# Autodesk Inventor assembly: KB33-046-001 - Ходовая часть
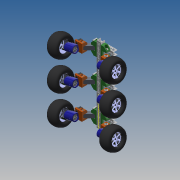
[picture p0: Inventor's stored thumbnail of the model, 180x180]
Saved by Autodesk Inventor 2020 (Build 240168000, 168)
## iProperties
Created: 2021-06-08
Part Number: KB33-046-001 - Ходовая часть
Material: Типовые
Document SubType Name: Assembly
Designer: Петров Иван
Mass: 8557.92 g
Surface Area: 14903.5 cm^2
Volume: 8211.85 cm^3
Density: 1.04214 g/cm^3
Author: Петров Иван
## Documents named in this file (6)
- E:\IVAN\Ivan_desktop\Kvantorium\Projects\RoboPatrol\design\KB33-046-002 - Рама.iam
- E:\IVAN\Ivan_desktop\Kvantorium\Projects\RoboPatrol\design\KB33-046-001-001 - Основание.ipt
- E:\IVAN\Ivan_desktop\Kvantorium\Projects\RoboPatrol\design\standart_components\Tetrix\ftc-tetrix-kit-of-parts-1.snapshot.34\MAX Channels\416mm Channel.ipt
- E:\IVAN\Ivan_desktop\Kvantorium\Projects\RoboPatrol\design\KB33-046-004 - Динамический модуль мотора в сборе.iam
- E:\IVAN\Ivan_desktop\Kvantorium\Projects\RoboPatrol\design\standart_components\Tetrix\ftc-tetrix-kit-of-parts-1.snapshot.34\MAX Channels\160mm Channel.ipt
- E:\IVAN\Ivan_desktop\Kvantorium\Projects\RoboPatrol\design\standart_components\Tetrix\ftc-tetrix-kit-of-parts-1.snapshot.34\Brackets\MAX Flat Bracket.ipt
## Components (14 placed, 5 different names)
1. KB33-046-001-001 - Основание:1
2. 416mm Channel:1 — Mate:1, Mate:2, Mate:3, Совмещение:4, Совмещение:8, Совмещение:9, Совмещение:10, Совмещение:11, Совмещение:13, Совмещение:14
3. 160mm Channel:1 — Совмещение:12, Совмещение:15, Совмещение:16, Совмещение:17
4. MAX Flat Bracket:1 — Совмещение:13, Совмещение:14, Совмещение:15
5. MAX Flat Bracket:2 — Совмещение:10, Совмещение:11, Совмещение:12
6. 160mm Channel:2 — Совмещение:16, Совмещение:17, Заподлицо:3
7. 160mm Channel:3
8. 160mm Channel:4
9. KB33-046-004 - Динамический модуль мотора в сборе:1 [sub-assembly] — Совмещение:4, Совмещение:8, Совмещение:9
10. KB33-046-004 - Динамический модуль мотора в сборе:2 [sub-assembly]
11. KB33-046-004 - Динамический модуль мотора в сборе:3 [sub-assembly] — Заподлицо:3
12. KB33-046-004 - Динамический модуль мотора в сборе:4 [sub-assembly]
13. KB33-046-004 - Динамический модуль мотора в сборе:5 [sub-assembly]
14. KB33-046-004 - Динамический модуль мотора в сборе:6 [sub-assembly]
## Component patterns: (2 elements), (3 elements, first: 160mm Channel:2), (3 elements, first: KB33-046-004 - Динамический модуль мотора в сборе:1), МассивКомп 6:2 (3 elements)
## Relationships (18: Mate 15, Flush 3)
- Mate:1: 416mm Channel:1
- Mate:2: 416mm Channel:1
- Mate:3: 416mm Channel:1
- Совмещение:4 [Mate]: 416mm Channel:1 ↔ KB33-046-004 - Динамический модуль мотора в сборе:1
- [Mate]: 416mm Channel:1 ↔ 160mm Channel:1
- [Flush]: 416mm Channel:1 ↔ 160mm Channel:1
- [Flush]: 416mm Channel:1 ↔ 160mm Channel:1
- Совмещение:8 [Mate]: 416mm Channel:1 ↔ KB33-046-004 - Динамический модуль мотора в сборе:1
- Совмещение:9 [Mate]: 416mm Channel:1 ↔ KB33-046-004 - Динамический модуль мотора в сборе:1
- Совмещение:10 [Mate]: 416mm Channel:1 ↔ MAX Flat Bracket:2
- Совмещение:11 [Mate]: 416mm Channel:1 ↔ MAX Flat Bracket:2
- Совмещение:12 [Mate]: 160mm Channel:1 ↔ MAX Flat Bracket:2
- Совмещение:13 [Mate]: 416mm Channel:1 ↔ MAX Flat Bracket:1
- Совмещение:14 [Mate]: 416mm Channel:1 ↔ MAX Flat Bracket:1
- Совмещение:15 [Mate]: 160mm Channel:1 ↔ MAX Flat Bracket:1
- Совмещение:16 [Mate]: 160mm Channel:1 ↔ 160mm Channel:2
- Совмещение:17 [Mate]: 160mm Channel:1 ↔ 160mm Channel:2
- Заподлицо:3 [Flush]: 160mm Channel:2 ↔ KB33-046-004 - Динамический модуль мотора в сборе:3
